# Autodesk Inventor assembly: InternalTopMoldAssembly
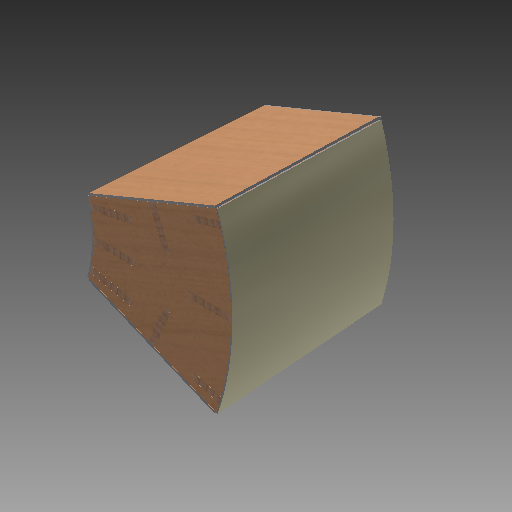
[picture p0: Inventor's stored thumbnail of the model, 512x512]
Saved by Autodesk Inventor 2019 (Build 230136000, 136)
## iProperties
Company: FABLAB Torino
Created: 2019-01-11
Part Number: InternalTopMoldAssembly
Document SubType Name: Assembly
Designer: Giancarlo
Project: La Panca - Flower Vase
Mass: 72304.3 g
Surface Area: 89186 cm^2
Volume: 48627 cm^3
Density: 1.48692 g/cm^3
Author: Giancarlo
Title: La Panca - Flower Vase
Subject: Construction MOld
## Documents named in this file (7)
- D:\Giancarlo Bacchio\Documenti\00 - Progetti\30-Inventor\flower vase\InternalTopMoldAssembly.iam
- D:\Giancarlo Bacchio\Documenti\00 - Progetti\30-Inventor\flower vase\intenalFormerTopAssembly.iam
- D:\Giancarlo Bacchio\Documenti\00 - Progetti\30-Inventor\flower vase\internalSupportTop1.ipt
- D:\Giancarlo Bacchio\Documenti\00 - Progetti\30-Inventor\flower vase\internalSupportTop2.ipt
- D:\Giancarlo Bacchio\Documenti\00 - Progetti\30-Inventor\flower vase\internalSupportTop3.ipt
- D:\Giancarlo Bacchio\Documenti\00 - Progetti\30-Inventor\flower vase\internalSupportTop4.ipt
- D:\Giancarlo Bacchio\Documenti\00 - Progetti\30-Inventor\flower vase\internalSupportTop5.ipt
## Components (11 placed, 6 different names)
1. internalSupportTop4:3 — Flush:58, Mate:1, Mate:2
2. internalSupportTop4:4 — Flush:60, Mate:3, Mate:4
3. internalSupportTop5:1 — Flush:56, Flush:57
4. internalSupportTop2:4 — Flush:59
5. internalSupportTop1:1 — Flush:42, Flush:43, Flush:58, Mate:1, Mate:2, Flush:59, Flush:60, Mate:3, Mate:4
6. internalSupportTop2:1
7. internalSupportTop3:1 — Flush:56, Flush:57
8. internalSupportTop3:2
9. internalSupportTop2:2
10. internalSupportTop2:3
11. intenalFormerTopAssembly:1 [sub-assembly] — Flush:42, Flush:43
## Relationships (11: Flush 7, Mate 4)
- Flush:42: internalSupportTop1:1 ↔ intenalFormerTopAssembly:1
- Flush:43: internalSupportTop1:1 ↔ intenalFormerTopAssembly:1
- Flush:56: internalSupportTop5:1 ↔ internalSupportTop3:1
- Flush:57: internalSupportTop5:1 ↔ internalSupportTop3:1
- Flush:58: internalSupportTop4:3 ↔ internalSupportTop1:1
- Mate:1: internalSupportTop4:3 ↔ internalSupportTop1:1
- Mate:2: internalSupportTop4:3 ↔ internalSupportTop1:1
- Flush:59: internalSupportTop2:4 ↔ internalSupportTop1:1
- Flush:60: internalSupportTop4:4 ↔ internalSupportTop1:1
- Mate:3: internalSupportTop4:4 ↔ internalSupportTop1:1
- Mate:4: internalSupportTop4:4 ↔ internalSupportTop1:1
